# Autodesk Inventor assembly: Tower
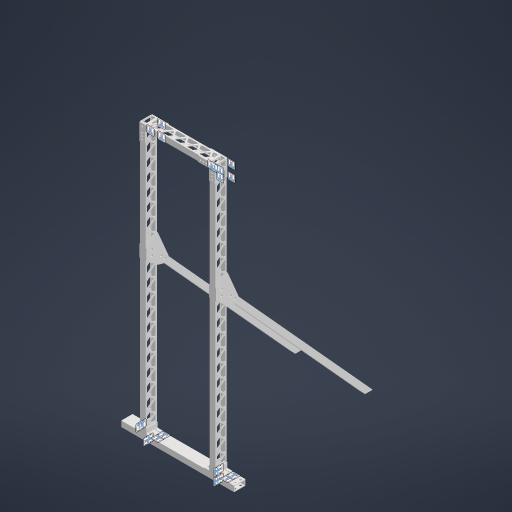
[picture p0: Inventor's stored thumbnail of the model, 512x512]
Saved by Autodesk Inventor 2023 (Build 270158000, 158)
## iProperties
Created: 2023-01-19
Part Number: Tower
Document SubType Name: Assembly
Designer: Terrence
Mass: 2797.17 g
Surface Area: 7389.26 cm^2
Volume: 1043.68 cm^3
Density: 2.6801 g/cm^3
Author: Terrence
## Documents named in this file (9)
- C:\Users\Terrence\Documents\FRC Long\Tower\Tower.iam
- C:\Users\Terrence\Documents\FRC Long\Tower\Solid1.ipt
- C:\Users\Terrence\Documents\FRC Long\Tower\Solid2.ipt
- C:\Users\Terrence\Documents\FRC Long\Tower\Solid3.ipt
- C:\Users\Terrence\Documents\FRC Long\Tower\Solid4.ipt
- C:\Users\Terrence\Documents\FRC Long\Tower\Solid6.ipt
- C:\Users\Terrence\Documents\FRC Long\Tower\Solid8.ipt
- C:\Users\Terrence\Documents\FRC Long\Tower\Solid7.ipt
- C:\Users\Terrence\Documents\FRC Long\Tower\Solid10.ipt
## Components (22 placed, 8 different names)
1. Solid1:1 — Insert:1, Insert:2, Insert:3, Insert:4, Insert:13, Insert:14, Insert:17, Insert:18, Insert:23, Insert:24, Insert:27, Insert:28
2. Solid2:1 — Insert:5, Insert:6, Insert:11, Insert:12
3. Solid3:1 — Insert:15, Insert:16, Insert:22
4. Solid4:1 — Insert:3, Insert:4, Insert:5, Insert:6
5. Solid4:2 — Insert:1, Insert:2
6. Solid4:4 — Insert:7, Insert:8, Insert:11, Insert:12
7. Solid1:2 — Insert:7, Insert:8, Insert:9, Insert:10, Insert:19, Insert:20, Insert:21, Insert:30, Insert:31, Insert:34
8. Solid4:5 — Insert:9, Insert:10
9. Solid6:1 — Insert:13, Insert:14, Insert:15, Insert:16
10. Solid6:2 — Insert:17, Insert:18
11. Solid6:3 — Insert:19, Insert:20
12. Solid6:4 — Insert:21, Insert:22
13. Solid8:1
14. Solid7:1 — Insert:25, Insert:26, Insert:29
15. Solid8:2
16. Solid8:3
17. Solid7:2 — Insert:32, Insert:33, Insert:35
18. Solid8:4
19. Solid10:1 — Insert:23, Insert:24, Insert:25, Insert:26
20. Solid10:2 — Insert:27, Insert:28, Insert:29
21. Solid10:3 — Insert:34, Insert:35
22. Solid10:4 — Insert:30, Insert:31, Insert:32, Insert:33
## Relationships (35: Insert 35)
- Insert:1: Solid1:1 ↔ Solid4:2
- Insert:2: Solid1:1 ↔ Solid4:2
- Insert:3: Solid1:1 ↔ Solid4:1
- Insert:4: Solid1:1 ↔ Solid4:1
- Insert:5: Solid2:1 ↔ Solid4:1
- Insert:6: Solid2:1 ↔ Solid4:1
- Insert:7: Solid4:4 ↔ Solid1:2
- Insert:8: Solid4:4 ↔ Solid1:2
- Insert:9: Solid1:2 ↔ Solid4:5
- Insert:10: Solid1:2 ↔ Solid4:5
- Insert:11: Solid2:1 ↔ Solid4:4
- Insert:12: Solid2:1 ↔ Solid4:4
- Insert:13: Solid1:1 ↔ Solid6:1
- Insert:14: Solid1:1 ↔ Solid6:1
- Insert:15: Solid3:1 ↔ Solid6:1
- Insert:16: Solid3:1 ↔ Solid6:1
- Insert:17: Solid1:1 ↔ Solid6:2
- Insert:18: Solid1:1 ↔ Solid6:2
- Insert:19: Solid1:2 ↔ Solid6:3
- Insert:20: Solid1:2 ↔ Solid6:3
- Insert:21: Solid1:2 ↔ Solid6:4
- Insert:22: Solid3:1 ↔ Solid6:4
- Insert:23: Solid1:1 ↔ Solid10:1
- Insert:24: Solid1:1 ↔ Solid10:1
- Insert:25: Solid7:1 ↔ Solid10:1
- Insert:26: Solid7:1 ↔ Solid10:1
- Insert:27: Solid1:1 ↔ Solid10:2
- Insert:28: Solid1:1 ↔ Solid10:2
- Insert:29: Solid7:1 ↔ Solid10:2
- Insert:30: Solid1:2 ↔ Solid10:4
- Insert:31: Solid1:2 ↔ Solid10:4
- Insert:32: Solid7:2 ↔ Solid10:4
- Insert:33: Solid7:2 ↔ Solid10:4
- Insert:34: Solid1:2 ↔ Solid10:3
- Insert:35: Solid7:2 ↔ Solid10:3
